# Autodesk Inventor assembly: Frame
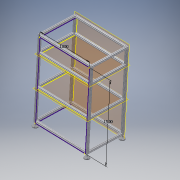
[picture p0: Inventor's stored thumbnail of the model, 180x180]
Saved by Autodesk Inventor 2016 (Build 200138000, 138)
## iProperties
Created: 2015-07-26
Part Number: Frame
Document SubType Name: Assembly
Designer: myhome
_SolveAssemblyDoc: Frame Generator Solve Assembly
_Version: 15.0.0
Author: myhome
## Documents named in this file (4)
- C:\Users\myhome\Documents\Inventor\Printer\Frame.iam
- C:\Users\myhome\Documents\Inventor\Printer\Part1.ipt
- C:\Users\myhome\Documents\Inventor\Printer\Frame\Frame\Frame0001.iam
- C:\Users\myhome\Documents\Inventor\Printer\21.1846 LEVELING FOOT M10 WITH BORES.iam
## Components (6 placed, 3 different names)
1. FrameSkeleton
2. Frame0001:1 [sub-assembly] — Rigid:1, Rigid:2, Rigid:3, Rigid:4
3. 21.1846 LEVELING FOOT M10 WITH BORES:1 [sub-assembly] — Rigid:3
4. 21.1846 LEVELING FOOT M10 WITH BORES:2 [sub-assembly] — Rigid:1
5. 21.1846 LEVELING FOOT M10 WITH BORES:4 [sub-assembly] — Rigid:2
6. 21.1846 LEVELING FOOT M10 WITH BORES:5 [sub-assembly] — Rigid:4
## Relationships (4: WeldJoint 4)
- Rigid:1 [WeldJoint]: Frame0001:1 ↔ 21.1846 LEVELING FOOT M10 WITH BORES:2
- Rigid:2 [WeldJoint]: Frame0001:1 ↔ 21.1846 LEVELING FOOT M10 WITH BORES:4
- Rigid:3 [WeldJoint]: Frame0001:1 ↔ 21.1846 LEVELING FOOT M10 WITH BORES:1
- Rigid:4 [WeldJoint]: Frame0001:1 ↔ 21.1846 LEVELING FOOT M10 WITH BORES:5
